# Autodesk Inventor assembly: SSE SiPM 8Ch_2026
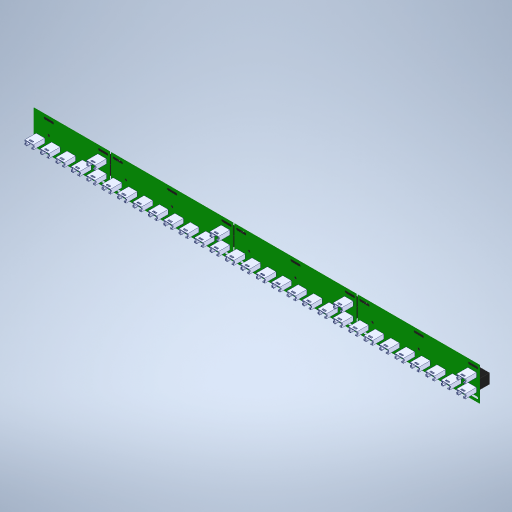
[picture p0: Inventor's stored thumbnail of the model, 512x512]
Saved by Autodesk Inventor 2024.2 (Build 282272000, 272)
## iProperties
Created: 2026-01-14
Part Number: SSE SiPM 8Ch_2026
Document SubType Name: Assembly
Designer: ja.restrepo1
Author: ja.restrepo1
## Documents named in this file (2)
- I:\MICROMECANICA\ALTAS ENERGIAS\Deteccion de Muones\Detectores centelladores\Partes Detector Centellador\SE Tarjetas IC DC\SSE SiPM 8Ch_2026.iam
- I:\MICROMECANICA\ALTAS ENERGIAS\Deteccion de Muones\Detectores centelladores\Partes Detector Centellador\SE Tarjetas IC DC\SiPM 8Ch V3_2026.iam
## Components (4 placed, 1 different names)
1. SiPM 8Ch V3_2026:1 [sub-assembly] — Flush:3, Flush:4, Mate:3, Mate:6
2. SiPM 8Ch V3_2026:2 [sub-assembly] — Flush:2, Flush:3, Flush:4, Flush:5, Mate:2, Mate:3
3. SiPM 8Ch V3_2026:3 [sub-assembly] — Flush:1, Flush:2, Flush:5, Flush:6, Mate:2
4. SiPM 8Ch V3_2026:4 [sub-assembly] — Flush:1, Flush:6, Mate:4, Flush:7, Mate:6, Mate:7
## Relationships (12: Flush 7, Mate 5)
- Flush:1: SiPM 8Ch V3_2026:3 ↔ SiPM 8Ch V3_2026:4
- Flush:2: SiPM 8Ch V3_2026:2 ↔ SiPM 8Ch V3_2026:3
- Flush:3: SiPM 8Ch V3_2026:1 ↔ SiPM 8Ch V3_2026:2
- Flush:4: SiPM 8Ch V3_2026:1 ↔ SiPM 8Ch V3_2026:2
- Flush:5: SiPM 8Ch V3_2026:2 ↔ SiPM 8Ch V3_2026:3
- Flush:6: SiPM 8Ch V3_2026:3 ↔ SiPM 8Ch V3_2026:4
- Mate:2 (2 mm): SiPM 8Ch V3_2026:2 ↔ SiPM 8Ch V3_2026:3
- Mate:3 (2 mm): SiPM 8Ch V3_2026:1 ↔ SiPM 8Ch V3_2026:2
- Mate:4: SiPM 8Ch V3_2026:4
- Flush:7 (-51 mm): SiPM 8Ch V3_2026:4
- Mate:6 (2 mm): SiPM 8Ch V3_2026:1 ↔ SiPM 8Ch V3_2026:4
- Mate:7 (-151.85 mm): SiPM 8Ch V3_2026:4
